# Autodesk Inventor assembly: ExoAssembly
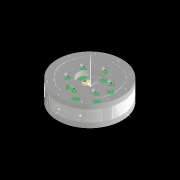
[picture p0: Inventor's stored thumbnail of the model, 180x180]
Saved by Autodesk Inventor 2022.2 (Build 262287010, 287A)
## iProperties
Created: 2022-06-03
Part Number: ExoAssembly
Document SubType Name: Assembly
Designer: Árni Þór Þorgeirsson
Author: Árni Þór Þorgeirsson
## Documents named in this file (6)
- G:\My Drive\Masters Thesis - exo\CAD_Files\ExoskeletonV0p2\ExoAssembly.iam
- G:\My Drive\Masters Thesis - exo\CAD_Files\ExoskeletonV0p2\OuterBearing_TBS\Left_OuterBearing_TBS.ipt
- G:\My Drive\Masters Thesis - exo\CAD_Files\External Hardware\Output_bearing_assembly.iam
- G:\My Drive\Masters Thesis - exo\CAD_Files\ExoskeletonV0p2\Rotor_TSB\PrintingTests\Printing_TestsRotor_TSB.ipt
- G:\My Drive\Masters Thesis - exo\CAD_Files\ExoskeletonV0p2\OuterBearing_TBS\Right_OuterBearing_TBS.ipt
- G:\My Drive\Masters Thesis - exo\CAD_Files\ExoskeletonV0p2\Stator_TSB\DriveGenerator_ParentFile.ipt
## Components (11 placed, 5 different names)
1. Left_OuterBearing_TBS:1 — Mate:1, Mate:2, Mate:3, Mate:5
2. Printing_TestsRotor_TSB:1 — Tangent:1, Tangent:2, Flush:1
3. Printing_TestsRotor_TSB:2 — Tangent:3, Tangent:4, Flush:2
4. Right_OuterBearing_TBS:1 — Mate:4, Insert:1, Insert:2, Cylindrical:1, Cylindrical:2
5. DriveGenerator_ParentFile:1 — Cylindrical:1, Cylindrical:2, Mate:5
6. Output_bearing_assembly:5 [sub-assembly] — Mate:1, Mate:2, Mate:3, Tangent:2, Tangent:4, Mate:4, Insert:2
7. Output_bearing_assembly:6 [sub-assembly] — Tangent:1, Flush:1, Tangent:3, Flush:2, Insert:1
8. Output_bearing_assembly:7 [sub-assembly]
9. Output_bearing_assembly:8 [sub-assembly]
10. Output_bearing_assembly:9 [sub-assembly]
11. Output_bearing_assembly:10 [sub-assembly]
## Component patterns: (6 elements, first: Output_bearing_assembly:5)
## Relationships (15: Mate 5, Tangent 4, Flush 2, Insert 2, CylindricalJoint 2)
- Mate:1: Left_OuterBearing_TBS:1 ↔ Output_bearing_assembly:5
- Mate:2: Left_OuterBearing_TBS:1 ↔ Output_bearing_assembly:5
- Mate:3: Left_OuterBearing_TBS:1 ↔ Output_bearing_assembly:5
- Tangent:1: Printing_TestsRotor_TSB:1 ↔ Output_bearing_assembly:6
- Tangent:2: Printing_TestsRotor_TSB:1 ↔ Output_bearing_assembly:5
- Flush:1: Printing_TestsRotor_TSB:1 ↔ Output_bearing_assembly:6
- Tangent:3: Printing_TestsRotor_TSB:2 ↔ Output_bearing_assembly:6
- Tangent:4: Printing_TestsRotor_TSB:2 ↔ Output_bearing_assembly:5
- Flush:2: Printing_TestsRotor_TSB:2 ↔ Output_bearing_assembly:6
- Mate:4: Right_OuterBearing_TBS:1 ↔ Output_bearing_assembly:5
- Insert:1: Right_OuterBearing_TBS:1 ↔ Output_bearing_assembly:6
- Insert:2: Right_OuterBearing_TBS:1 ↔ Output_bearing_assembly:5
- Cylindrical:1: Right_OuterBearing_TBS:1 ↔ DriveGenerator_ParentFile:1
- Cylindrical:2: Right_OuterBearing_TBS:1 ↔ DriveGenerator_ParentFile:1
- Mate:5: Left_OuterBearing_TBS:1 ↔ DriveGenerator_ParentFile:1
